# Autodesk Inventor assembly: OnyxBody
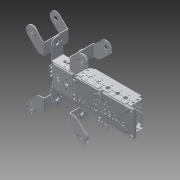
[picture p0: Inventor's stored thumbnail of the model, 180x180]
Saved by Autodesk Inventor 2015 (Build 190159000, 159)
## iProperties
Created: 2015-05-21
Part Number: OnyxBody
Document SubType Name: Assembly
Designer: Quinn
Author: Quinn
## Documents named in this file (25)
- C:\Users\Quinn\Desktop\3DCNC Design\InventorModels\Assemblies\OnyxBody.iam
- C:\Users\Quinn\Desktop\3DCNC Design\InventorModels\Metal\Brackets\asb-12-StandardCChannel.ipt
- C:\Users\Quinn\Desktop\3DCNC Design\InventorModels\Metal\Brackets\asb-06-LTab.ipt
- C:\Users\Quinn\Desktop\3DCNC Design\InventorModels\Metal\Brackets\asb-09-StandardC.ipt
- C:\Users\Quinn\Desktop\3DCNC Design\InventorModels\Metal\Brackets\asb-15-MulitPurpose.ipt
- C:\Users\Quinn\Desktop\3DCNC Design\InventorModels\Plastics\RearCarriageSupport.ipt
- C:\Users\Quinn\Desktop\3DCNC Design\InventorModels\Plastics\RearCarriageCarrierPlate.ipt
- C:\Users\Quinn\Desktop\3DCNC Design\InventorModels\Metal\Brackets\asb-11-angleC.ipt
- C:\Users\Quinn\Desktop\3DCNC Design\InventorModels\Plastics\OnxyBelly.ipt
- C:\Users\Quinn\Desktop\3DCNC Design\InventorModels\Assemblies\OnyxBody\Design Accelerator\Bolted Connection1.iam
- C:\Users\Quinn\Desktop\3DCNC Design\InventorModels\Assemblies\OnyxBody\Design Accelerator\Bolted Connection2.iam
- C:\Users\Quinn\Desktop\3DCNC Design\InventorModels\Assemblies\OnyxBody\Design Accelerator\Bolted Connection3.iam
- C:\Users\Quinn\Desktop\3DCNC Design\InventorModels\Assemblies\OnyxBody\Design Accelerator\Bolted Connection4.iam
- C:\Users\Quinn\Desktop\3DCNC Design\InventorModels\Assemblies\OnyxBody\Design Accelerator\Bolted Connection5.iam
- C:\Users\Quinn\Desktop\3DCNC Design\InventorModels\Assemblies\OnyxBody\Design Accelerator\Bolted Connection6.iam
- C:\Users\Quinn\Desktop\3DCNC Design\InventorModels\Electronics\Servo\ServoHornPlastic.ipt
- C:\Users\Quinn\Desktop\3DCNC Design\InventorModels\Assemblies\OnyxBody\Design Accelerator\Bolted Connection7.iam
- C:\Users\Quinn\Desktop\3DCNC Design\InventorModels\Assemblies\OnyxBody\Design Accelerator\Bolted Connection8.iam
- C:\Users\Quinn\Desktop\3DCNC Design\InventorModels\Assemblies\OnyxBody\Design Accelerator\Bolted Connection9.iam
- C:\Users\Quinn\Desktop\3DCNC Design\InventorModels\Assemblies\OnyxBody\Design Accelerator\Bolted Connection10.iam
- C:\Users\Quinn\Desktop\3DCNC Design\InventorModels\Assemblies\OnyxBody\Design Accelerator\Bolted Connection11.iam
- C:\Users\Quinn\Desktop\3DCNC Design\InventorModels\Assemblies\OnyxBody\Design Accelerator\Bolted Connection12.iam
- C:\Users\Quinn\Desktop\3DCNC Design\InventorModels\Assemblies\OnyxBody\Design Accelerator\Bolted Connection13.iam
- C:\Users\Quinn\Desktop\3DCNC Design\InventorModels\Assemblies\OnyxBody\Design Accelerator\Bolted Connection14.iam
- C:\Users\Quinn\Desktop\3DCNC Design\InventorModels\Assemblies\OnyxBody\Design Accelerator\Bolted Connection15.iam
## Components (33 placed, 10 different names)
1. asb-12-StandardCChannel:1 — Mate:1, Mate:5, Mate:6, Mate:24, Mate:53, Mate:54
2. asb-06-LTab:1 — Mate:1, Mate:2, Mate:47, Mate:48
3. asb-09-StandardC:2 — Mate:2, Mate:3, Mate:4
4. asb-15-MulitPurpose:1 — Mate:4, Mate:7, Mate:8
5. asb-15-MulitPurpose:2 — Mate:3
6. asb-09-StandardC:3 — Mate:5, Mate:11, Mate:12, Mate:27, Mate:28
7. asb-09-StandardC:4 — Mate:6, Mate:9, Mate:10, Mate:25, Mate:26
8. RearCarriageSupport:1 — Mate:7, Mate:49, Mate:50, Mate:51, Mate:52
9. RearCarriageCarrierPlate:1 — Mate:8, Mate:45, Mate:46
10. asb-11-angleC:1 — Mate:11, Mate:33, Mate:34, Insert:3, Mate:37, Mate:38
11. asb-11-angleC:2 — Mate:12, Mate:35, Mate:36, Insert:4, Mate:43, Mate:44
12. asb-11-angleC:3 — Mate:9, Mate:31, Mate:32, Insert:1, Mate:41, Mate:42
13. asb-11-angleC:4 — Mate:10, Mate:29, Mate:30, Insert:2, Mate:39, Mate:40
14. OnxyBelly:1 — Mate:24
15. Bolted Connection:1 [sub-assembly] — Mate:25, Mate:26
16. Bolted Connection:2 [sub-assembly] — Mate:27, Mate:28
17. Bolted Connection:3 [sub-assembly] — Mate:29, Mate:30
18. Bolted Connection:4 [sub-assembly] — Mate:31, Mate:32
19. Bolted Connection:5 [sub-assembly] — Mate:33, Mate:34
20. Bolted Connection:6 [sub-assembly] — Mate:35, Mate:36
21. ServoHornPlastic:1 — Insert:1
22. ServoHornPlastic:2 — Insert:4
23. ServoHornPlastic:3 — Insert:3
24. ServoHornPlastic:4 — Insert:2
25. Bolted Connection:7 [sub-assembly] — Mate:37, Mate:38
26. Bolted Connection:8 [sub-assembly] — Mate:39, Mate:40
27. Bolted Connection:9 [sub-assembly] — Mate:41, Mate:42
28. Bolted Connection:10 [sub-assembly] — Mate:43, Mate:44
29. Bolted Connection:11 [sub-assembly] — Mate:45, Mate:46
30. Bolted Connection:12 [sub-assembly] — Mate:47, Mate:48
31. Bolted Connection:13 [sub-assembly] — Mate:49, Mate:50
32. Bolted Connection:14 [sub-assembly] — Mate:51, Mate:52
33. Bolted Connection:15 [sub-assembly] — Mate:53, Mate:54
## Relationships (47: Mate 43, Insert 4)
- Mate:1: asb-12-StandardCChannel:1 ↔ asb-06-LTab:1
- Mate:2: asb-06-LTab:1 ↔ asb-09-StandardC:2
- Mate:3: asb-09-StandardC:2 ↔ asb-15-MulitPurpose:2
- Mate:4: asb-09-StandardC:2 ↔ asb-15-MulitPurpose:1
- Mate:5: asb-12-StandardCChannel:1 ↔ asb-09-StandardC:3
- Mate:6: asb-12-StandardCChannel:1 ↔ asb-09-StandardC:4
- Mate:7: asb-15-MulitPurpose:1 ↔ RearCarriageSupport:1
- Mate:8: asb-15-MulitPurpose:1 ↔ RearCarriageCarrierPlate:1
- Mate:9: asb-09-StandardC:4 ↔ asb-11-angleC:3
- Mate:10: asb-09-StandardC:4 ↔ asb-11-angleC:4
- Mate:11: asb-09-StandardC:3 ↔ asb-11-angleC:1
- Mate:12: asb-09-StandardC:3 ↔ asb-11-angleC:2
- Mate:24: asb-12-StandardCChannel:1 ↔ OnxyBelly:1
- Mate:25: asb-09-StandardC:4 ↔ Bolted Connection:1
- Mate:26: asb-09-StandardC:4 ↔ Bolted Connection:1
- Mate:27: asb-09-StandardC:3 ↔ Bolted Connection:2
- Mate:28: asb-09-StandardC:3 ↔ Bolted Connection:2
- Mate:29: asb-11-angleC:4 ↔ Bolted Connection:3
- Mate:30: asb-11-angleC:4 ↔ Bolted Connection:3
- Mate:31: asb-11-angleC:3 ↔ Bolted Connection:4
- Mate:32: asb-11-angleC:3 ↔ Bolted Connection:4
- Mate:33: asb-11-angleC:1 ↔ Bolted Connection:5
- Mate:34: asb-11-angleC:1 ↔ Bolted Connection:5
- Mate:35: asb-11-angleC:2 ↔ Bolted Connection:6
- Mate:36: asb-11-angleC:2 ↔ Bolted Connection:6
- Insert:1: asb-11-angleC:3 ↔ ServoHornPlastic:1
- Insert:2: asb-11-angleC:4 ↔ ServoHornPlastic:4
- Insert:3: asb-11-angleC:1 ↔ ServoHornPlastic:3
- Insert:4: asb-11-angleC:2 ↔ ServoHornPlastic:2
- Mate:37: asb-11-angleC:1 ↔ Bolted Connection:7
- Mate:38: asb-11-angleC:1 ↔ Bolted Connection:7
- Mate:39: asb-11-angleC:4 ↔ Bolted Connection:8
- Mate:40: asb-11-angleC:4 ↔ Bolted Connection:8
- Mate:41: asb-11-angleC:3 ↔ Bolted Connection:9
- Mate:42: asb-11-angleC:3 ↔ Bolted Connection:9
- Mate:43: asb-11-angleC:2 ↔ Bolted Connection:10
- Mate:44: asb-11-angleC:2 ↔ Bolted Connection:10
- Mate:45: RearCarriageCarrierPlate:1 ↔ Bolted Connection:11
- Mate:46: RearCarriageCarrierPlate:1 ↔ Bolted Connection:11
- Mate:47: asb-06-LTab:1 ↔ Bolted Connection:12
- Mate:48: asb-06-LTab:1 ↔ Bolted Connection:12
- Mate:49: RearCarriageSupport:1 ↔ Bolted Connection:13
- Mate:50: RearCarriageSupport:1 ↔ Bolted Connection:13
- Mate:51: RearCarriageSupport:1 ↔ Bolted Connection:14
- Mate:52: RearCarriageSupport:1 ↔ Bolted Connection:14
- Mate:53: asb-12-StandardCChannel:1 ↔ Bolted Connection:15
- Mate:54: asb-12-StandardCChannel:1 ↔ Bolted Connection:15
